# Autodesk Inventor assembly: LCD
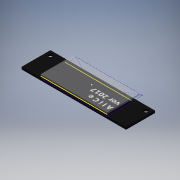
[picture p0: Inventor's stored thumbnail of the model, 180x180]
Saved by Autodesk Inventor 2016 (Build 200138000, 138)
## iProperties
Created: 2017-06-12
Part Number: LCD
Material: 一般
Document SubType Name: Assembly
Designer: B4_Ohno
Author: B4_Ohno
## Documents named in this file (4)
- C:\Users\B4_Ohno\Dropbox\AliCe関連\MicroMouse2016\LCD.iam
- C:\Users\B4_Ohno\Dropbox\AliCe関連\MicroMouse2016\kiban.ipt
- C:\Users\B4_Ohno\Dropbox\AliCe関連\MicroMouse2016\monitor.ipt
- C:\Users\B4_Ohno\Dropbox\AliCe関連\MicroMouse2016\panel.ipt
## Components (3 placed, 3 different names)
1. kiban:1 — フラッシュ:3
2. monitor:1 — フラッシュ:2, フラッシュ:3
3. panel:1 — フラッシュ:2
## Relationships (2: Flush 2)
- フラッシュ:2 [Flush]: monitor:1 ↔ panel:1
- フラッシュ:3 [Flush]: kiban:1 ↔ monitor:1
